# Autodesk Inventor assembly: Assy_cam_connection
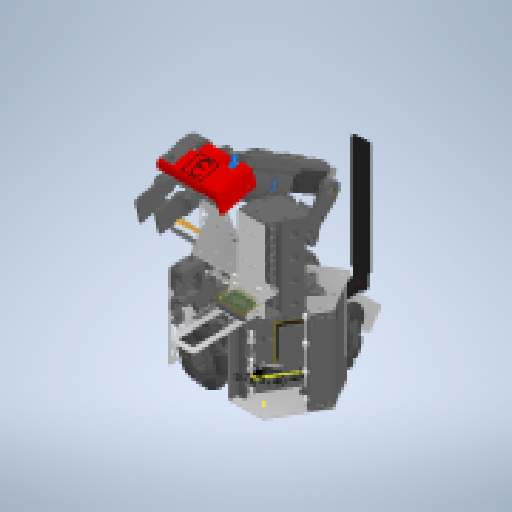
[picture p0: Inventor's stored thumbnail of the model, 512x512]
Saved by Autodesk Inventor 2024.1 (Build 281209000, 209)
## iProperties
Created: 2025-03-04
Part Number: Assy_cam_connection
Document SubType Name: Assembly
Designer: hibik
Author: hibik
## Documents named in this file (7)
- C:\Users\hibik\Documents\Robomech\RESCUE\ORCA\hard\Assy_cam_connection.iam
- C:\Users\hibik\Documents\Robomech\RESCUE\ORCA\hard\Assy_fork_connection.iam
- C:\Users\hibik\Documents\Robomech\RESCUE\ORCA\hard\flame_front\cam_setter_left_under.ipt
- C:\Users\hibik\Documents\Robomech\RESCUE\ORCA\hard\flame_front\cam_setter_left_upper.ipt
- C:\Users\hibik\Documents\Robomech\RESCUE\ORCA\hard\flame_front\cam_setter_right_under.ipt
- C:\Users\hibik\Documents\Robomech\RESCUE\ORCA\hard\flame_front\cam_setter_right_upper.ipt
- C:\Users\hibik\Documents\Robomech\RESCUE\ORCA\hard\arm\Assy_arm.iam
## Components (6 placed, 6 different names)
1. Assy_fork_connection:1 [sub-assembly] — 挿入:11, 挿入:12, 挿入:17, 挿入:18
2. cam_setter_left_under:1 — 挿入:11, 挿入:15
3. cam_setter_left_upper:1 — 挿入:16
4. cam_setter_right_under:1 — 挿入:12, 挿入:16
5. cam_setter_right_upper:1 — 挿入:15
6. Assy_arm:1 [sub-assembly] — 挿入:17, 挿入:18
## Relationships (6: Insert 6)
- 挿入:11 [Insert]: Assy_fork_connection:1 ↔ cam_setter_left_under:1
- 挿入:12 [Insert]: Assy_fork_connection:1 ↔ cam_setter_right_under:1
- 挿入:15 [Insert]: cam_setter_left_under:1 ↔ cam_setter_right_upper:1
- 挿入:16 [Insert]: cam_setter_left_upper:1 ↔ cam_setter_right_under:1
- 挿入:17 [Insert]: Assy_fork_connection:1 ↔ Assy_arm:1
- 挿入:18 [Insert]: Assy_fork_connection:1 ↔ Assy_arm:1
